# Autodesk Inventor assembly: RC V1
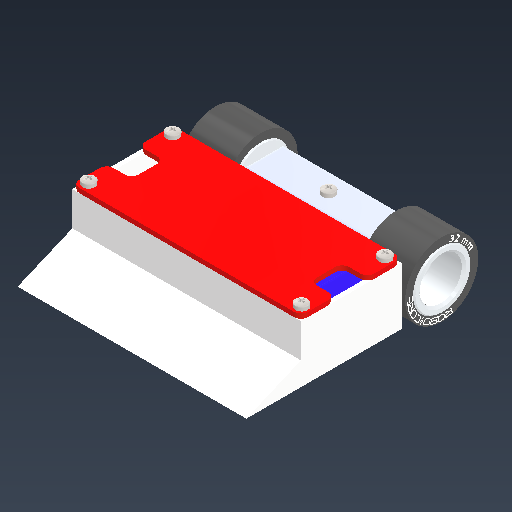
[picture p0: Inventor's stored thumbnail of the model, 512x512]
Saved by Autodesk Inventor 2026.1 (Build 301233020, 233B)
## iProperties
Created: 2025-07-10
Part Number: RC V1
Description: STEP AP214
Document SubType Name: Assembly
Designer: celio
Sending System: SolidWorks 2023
Preprocessor: SwSTEP 2.0
Title: RC V1.STEP
Revision Number: ANY
## Documents named in this file (9)
- C:\Users\celio\OneDrive\Documentos\Minisumo\minisumo-rc-1.snapshot.21\RC V1\RC V1\RC V1.iam
- C:\Users\celio\OneDrive\Documentos\Minisumo\minisumo-rc-1.snapshot.21\RC V1\RC V1\Chasis v1.ipt
- C:\Users\celio\OneDrive\Documentos\Minisumo\minisumo-rc-1.snapshot.21\RC V1\RC V1\Tapa Chasis.ipt
- C:\Users\celio\OneDrive\Documentos\Minisumo\minisumo-rc-1.snapshot.21\RC V1\RC V1\BATERIA.ipt
- C:\Users\celio\OneDrive\Documentos\Minisumo\minisumo-rc-1.snapshot.21\RC V1\RC V1\pan cross head_am_B18.6.7M - M3 x 0.5 x 6 Type I Cross Recessed PHMS --6N.ipt
- C:\Users\celio\OneDrive\Documentos\Minisumo\minisumo-rc-1.snapshot.21\RC V1\RC V1\Tapa Motor v1.ipt
- C:\Users\celio\OneDrive\Documentos\Minisumo\minisumo-rc-1.snapshot.21\RC V1\RC V1\PCB Redboard v2.iam
- C:\Users\celio\OneDrive\Documentos\Inventor\ZeGuia\Motores\N20\N20 DC MOTOR.ipt
- C:\Users\celio\OneDrive\Documentos\Minisumo\stickymax-silicone-wheel-32mm-v1-1-1.snapshot.7\Roda_StickyMAX-32mm-V1-1\Roda_StickyMAX-32mm-V1-1\Roda_StickyMAX-32mm-V1-1.iam
## Components (14 placed, 12 different names)
1. Chasis v1_1 — Coincidente:1, Coincidente:2, Coincidente:3, Coincidente:5, Coincidente:6, Coincidente:7, Coincidente:8, Coincidente:9
2. Tapa Chasis_4
3. BATERIA_7
4. pan cross head_am_B18.6.7M - M3 x 0.5 x 6 Type I Cross Recessed PHMS --6N_10
5. pan cross head_am_B18.6.7M - M3 x 0.5 x 6 Type I Cross Recessed PHMS --6N_11
6. pan cross head_am_B18.6.7M - M3 x 0.5 x 6 Type I Cross Recessed PHMS --6N_12
7. pan cross head_am_B18.6.7M - M3 x 0.5 x 6 Type I Cross Recessed PHMS --6N_13
8. pan cross head_am_B18.6.7M - M3 x 0.5 x 6 Type I Cross Recessed PHMS --6N_14
9. Tapa Motor v1_15
10. PCB Redboard v2_16 [sub-assembly]
11. N20 DC MOTOR:1 — Coincidente:1, Coincidente:2, Coincidente:3, Coincidente:4
12. Roda_StickyMAX-32mm-V1-1:1 [sub-assembly] — Coincidente:4, Coincidente:5
13. N20 DC MOTOR:2 — Coincidente:6, Coincidente:7, Coincidente:8, Coincidente:10
14. Roda_StickyMAX-32mm-V1-1:2 [sub-assembly] — Coincidente:9, Coincidente:10
## Relationships (10: Mate 10)
- Coincidente:1 [Mate]: Chasis v1_1 ↔ N20 DC MOTOR:1
- Coincidente:2 [Mate]: Chasis v1_1 ↔ N20 DC MOTOR:1
- Coincidente:3 [Mate]: Chasis v1_1 ↔ N20 DC MOTOR:1
- Coincidente:4 [Mate]: N20 DC MOTOR:1 ↔ Roda_StickyMAX-32mm-V1-1:1
- Coincidente:5 [Mate]: Chasis v1_1 ↔ Roda_StickyMAX-32mm-V1-1:1
- Coincidente:6 [Mate]: Chasis v1_1 ↔ N20 DC MOTOR:2
- Coincidente:7 [Mate]: Chasis v1_1 ↔ N20 DC MOTOR:2
- Coincidente:8 [Mate]: Chasis v1_1 ↔ N20 DC MOTOR:2
- Coincidente:9 [Mate]: Chasis v1_1 ↔ Roda_StickyMAX-32mm-V1-1:2
- Coincidente:10 [Mate]: N20 DC MOTOR:2 ↔ Roda_StickyMAX-32mm-V1-1:2
